# Autodesk Inventor assembly: Outer_C_Channel_30_MIR
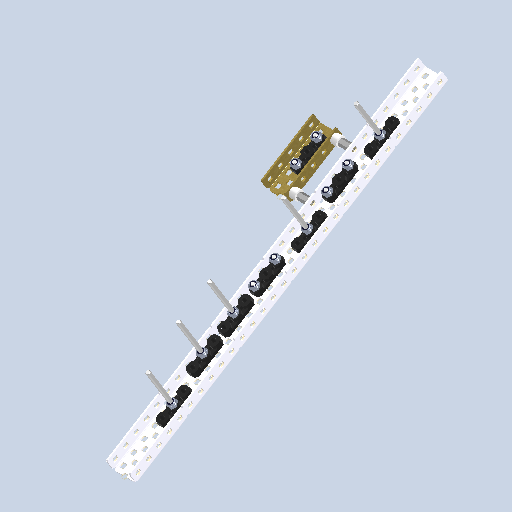
[picture p0: Inventor's stored thumbnail of the model, 512x512]
Saved by Autodesk Inventor 2025.2 (Build 292293000, 293)
## iProperties
Created: 2024-12-08
Part Number: Outer_C_Channel_30_MIR
Document SubType Name: Assembly
Designer: joshi
Author: Aditya Koduri
## Documents named in this file (12)
- C:\Users\joshi\Desktop\3388K CAD\Outer_C_Channel_30_MIR.iam
- C:\Users\joshi\Desktop\3388K CAD\VEX Main\Structure\C Channel\Aluminum 1x2x1\Alu C 1x2x1x30_MIR.ipt
- C:\Users\joshi\Desktop\3388K CAD\VEX Main\Motion\Shaft LS\Bearing Flat_MIR.ipt
- C:\Users\joshi\Desktop\3388K CAD\Screw_Joint_MIR.iam
- C:\Users\joshi\Desktop\3388K CAD\VEX Main\Structure\C Channel\Aluminum 1x2x1\Alu C 1x2x1x5_MIR.ipt
- C:\Users\joshi\Desktop\3388K CAD\VEX Main\Motion\Spacers\Spacer Nylon .313 OD\NSpacer .313 OD x .250.ipt
- C:\Users\joshi\Desktop\3388K CAD\VEX Main\Motion\Spacers\Spacer Nylon .313 OD.ipt
- C:\Users\joshi\Desktop\3388K CAD\VEX Main\Structure\Standoff\Standoff .50.ipt
- C:\Users\joshi\Desktop\3388K CAD\VEX Main\Structure\Standoff.ipt
- C:\Users\joshi\Desktop\3388K CAD\VEX Main\Structure\Hardware\Nut Thin Nylock_MIR.ipt
- C:\Users\joshi\Desktop\3388K CAD\VEX Main\Structure\Hardware\Screw Steel - Hex\SScrew Hex Smooth .500.ipt
- C:\Users\joshi\Desktop\3388K CAD\VEX Main\Structure\Hardware\Screw Steel - Hex.ipt
## Components (26 placed, 8 different names)
1. Alu C 1x2x1x30_MIR:1 — Insert:101, Insert:100, Insert:85, Insert:86, Insert:87, Insert:94, Insert:93, Insert:99, Insert:98, Insert:95, Insert:107, Insert:104, Insert:105, Insert:106, Insert:114
2. Bearing Flat_MIR:1 — Insert:97, Insert:96, Insert:111, Insert:110
3. Bearing Flat_MIR:2 — Insert:101, Insert:100, Insert:113, Insert:112
4. Screw_Joint_MIR:1 [sub-assembly] — Insert:85
5. Screw_Joint_MIR:2 [sub-assembly] — Insert:86
6. Screw_Joint_MIR:3 [sub-assembly] — Insert:87
7. Alu C 1x2x1x5_MIR:1 — Insert:97, Insert:96, Insert:89, Insert:90, Insert:102, Insert:103
8. NSpacer .313 OD x .250:1 — Insert:89, Insert:92
9. NSpacer .313 OD x .250:2 — Insert:90, Insert:91
10. Standoff .50:1 — Insert:94, Insert:91
11. Standoff .50:2 — Insert:93, Insert:92
12. Bearing Flat_MIR:3 — Insert:99, Insert:98, Insert:108, Insert:109
13. Screw_Joint_MIR:4 [sub-assembly] — Insert:95
14. Nut Thin Nylock_MIR:1 — Insert:113
15. Nut Thin Nylock_MIR:2 — Insert:112
16. SScrew Hex Smooth .500:1 — Insert:102
17. SScrew Hex Smooth .500:2 — Insert:107
18. Nut Thin Nylock_MIR:3 — Insert:108
19. Nut Thin Nylock_MIR:4 — Insert:111
20. SScrew Hex Smooth .500:3 — Insert:104
21. SScrew Hex Smooth .500:4 — Insert:105
22. Nut Thin Nylock_MIR:5 — Insert:109
23. Nut Thin Nylock_MIR:6 — Insert:110
24. SScrew Hex Smooth .500:5 — Insert:103
25. SScrew Hex Smooth .500:6 — Insert:106
26. Screw_Joint_MIR:5 [sub-assembly] — Insert:114
## Relationships (29: Insert 29)
- Insert:101: Alu C 1x2x1x30_MIR:1 ↔ Bearing Flat_MIR:2
- Insert:100: Alu C 1x2x1x30_MIR:1 ↔ Bearing Flat_MIR:2
- Insert:85: Alu C 1x2x1x30_MIR:1 ↔ Screw_Joint_MIR:1
- Insert:86: Alu C 1x2x1x30_MIR:1 ↔ Screw_Joint_MIR:2
- Insert:87: Alu C 1x2x1x30_MIR:1 ↔ Screw_Joint_MIR:3
- Insert:97: Bearing Flat_MIR:1 ↔ Alu C 1x2x1x5_MIR:1
- Insert:96: Bearing Flat_MIR:1 ↔ Alu C 1x2x1x5_MIR:1
- Insert:89: Alu C 1x2x1x5_MIR:1 ↔ NSpacer .313 OD x .250:1
- Insert:90: Alu C 1x2x1x5_MIR:1 ↔ NSpacer .313 OD x .250:2
- Insert:94: Alu C 1x2x1x30_MIR:1 ↔ Standoff .50:1
- Insert:91: NSpacer .313 OD x .250:2 ↔ Standoff .50:1
- Insert:93: Alu C 1x2x1x30_MIR:1 ↔ Standoff .50:2
- Insert:92: NSpacer .313 OD x .250:1 ↔ Standoff .50:2
- Insert:99: Alu C 1x2x1x30_MIR:1 ↔ Bearing Flat_MIR:3
- Insert:98: Alu C 1x2x1x30_MIR:1 ↔ Bearing Flat_MIR:3
- Insert:95: Alu C 1x2x1x30_MIR:1 ↔ Screw_Joint_MIR:4
- Insert:113: Bearing Flat_MIR:2 ↔ Nut Thin Nylock_MIR:1
- Insert:112: Bearing Flat_MIR:2 ↔ Nut Thin Nylock_MIR:2
- Insert:102: Alu C 1x2x1x5_MIR:1 ↔ SScrew Hex Smooth .500:1
- Insert:107: Alu C 1x2x1x30_MIR:1 ↔ SScrew Hex Smooth .500:2
- Insert:108: Bearing Flat_MIR:3 ↔ Nut Thin Nylock_MIR:3
- Insert:111: Bearing Flat_MIR:1 ↔ Nut Thin Nylock_MIR:4
- Insert:104: Alu C 1x2x1x30_MIR:1 ↔ SScrew Hex Smooth .500:3
- Insert:105: Alu C 1x2x1x30_MIR:1 ↔ SScrew Hex Smooth .500:4
- Insert:109: Bearing Flat_MIR:3 ↔ Nut Thin Nylock_MIR:5
- Insert:110: Bearing Flat_MIR:1 ↔ Nut Thin Nylock_MIR:6
- Insert:103: Alu C 1x2x1x5_MIR:1 ↔ SScrew Hex Smooth .500:5
- Insert:106: Alu C 1x2x1x30_MIR:1 ↔ SScrew Hex Smooth .500:6
- Insert:114: Alu C 1x2x1x30_MIR:1 ↔ Screw_Joint_MIR:5
